# Autodesk Inventor assembly: Assembled
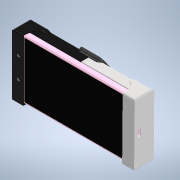
[picture p0: Inventor's stored thumbnail of the model, 180x180]
Saved by Autodesk Inventor 2020 (Build 240168000, 168)
## iProperties
Created: 2020-12-04
Part Number: Assembled
Document SubType Name: Assembly
Designer: Curtis
Author: Curtis
## Documents named in this file (10)
- D:\CAD\leeco-freon\Assembled-noEONpcb.iam
- D:\CAD\leeco-freon\heatsink.ipt
- D:\CAD\leeco-freon\leeco.ipt
- D:\CAD\leeco-freon\printed parts\28degree go pro mount.ipt
- D:\CAD\leeco-freon\printed parts\bottomclip.ipt
- D:\CAD\leeco-freon\printed parts\fanduct2.ipt
- D:\CAD\leeco-freon\printed parts\left.ipt
- D:\CAD\leeco-freon\printed parts\windshield mount.ipt
- D:\CAD\leeco-freon\noctua fan\NF-A4x10_Noctua_40mm.iam
- D:\CAD\leeco-freon\printed parts\right-noEONpcb.ipt
## Components (9 placed, 9 different names)
1. heatsink:1 — Mate:6, Flush:3, Mate:24
2. leeco:1 — Mate:4, Mate:6, Flush:3, Mate:8, Mate:22, Mate:23
3. 28degree go pro mount:1 — Mate:14, Mate:18, Mate:19, Mate:20
4. bottomclip:1 — Mate:16
5. fanduct2:1 — Mate:8, Mate:12, Mate:13
6. left:1 — Mate:4, Mate:14, Mate:16, Mate:24
7. windshield mount:1 — Mate:18, Mate:19, Mate:20
8. NF-A4x10_Noctua_40mm:1 [sub-assembly] — Mate:12, Mate:13
9. right-noEONpcb:1 — Mate:22, Mate:23
## Relationships (14: Mate 13, Flush 1)
- Mate:4: leeco:1 ↔ left:1
- Mate:6: heatsink:1 ↔ leeco:1
- Flush:3 (7 mm): heatsink:1 ↔ leeco:1
- Mate:8: leeco:1 ↔ fanduct2:1
- Mate:12: fanduct2:1 ↔ NF-A4x10_Noctua_40mm:1
- Mate:13: fanduct2:1 ↔ NF-A4x10_Noctua_40mm:1
- Mate:14: 28degree go pro mount:1 ↔ left:1
- Mate:16: bottomclip:1 ↔ left:1
- Mate:18: 28degree go pro mount:1 ↔ windshield mount:1
- Mate:19 (0.1 mm): 28degree go pro mount:1 ↔ windshield mount:1
- Mate:20: 28degree go pro mount:1 ↔ windshield mount:1
- Mate:22: leeco:1 ↔ right-noEONpcb:1
- Mate:23: leeco:1 ↔ right-noEONpcb:1
- Mate:24: heatsink:1 ↔ left:1
